# Autodesk Inventor assembly: Cover_Event_asm
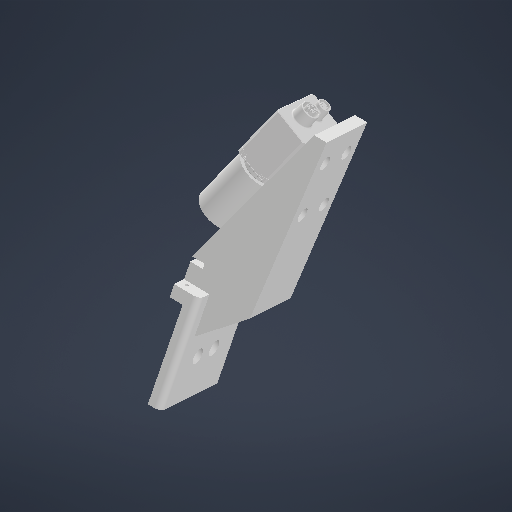
[picture p0: Inventor's stored thumbnail of the model, 512x512]
Saved by Autodesk Inventor 2026 (Build 300175000, 175)
## iProperties
Created: 2025-04-20
Part Number: Cover_Event_asm
Document SubType Name: Assembly
Designer: Charl
Author: Charl
## Documents named in this file (3)
- C:\School\Research\Inventor\v0.3\Cover\Cover_Event_asm.iam
- C:\School\Research\Inventor\v0.3\Cover\Camera_Bracket_Uru_001.ipt
- C:\School\Research\Inventor\v0.3\Camera\Triton2_asm.iam
## Components (2 placed, 2 different names)
1. Camera_Bracket_Uru_001:1 — Mate:1, Mate:2
2. Triton2_asm:1 [sub-assembly] — Mate:1, Mate:2
## Relationships (2: Mate 2)
- Mate:1: Camera_Bracket_Uru_001:1 ↔ Triton2_asm:1
- Mate:2: Camera_Bracket_Uru_001:1 ↔ Triton2_asm:1
